# Autodesk Inventor assembly: -ZPanel
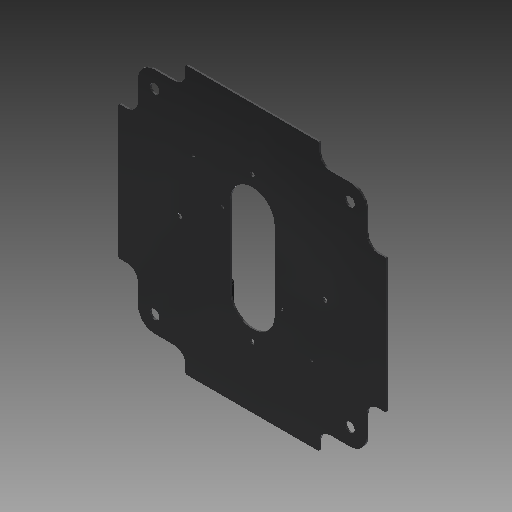
[picture p0: Inventor's stored thumbnail of the model, 512x512]
Saved by Autodesk Inventor 2018 (Build 220112000, 112)
## iProperties
Created: 2018-11-03
Part Number: -ZPanel
Document SubType Name: Assembly
Designer: Bradley
Author: Bradley
## Documents named in this file (3)
- C:\Users\Bradley\Documents\GitHub\CougSat1-Hardware\CougSat1-RadioBoard\CADModel\Native\-ZPanel.iam
- C:\Users\Bradley\Documents\GitHub\CougSat1-Hardware\CougSat1-RadioBoard\CADModel\Native\-ZPanel_PCB.ipt
- C:\Users\Bradley\Documents\GitHub\Resources\SupplierDocuments\04 - Connectors SMT\04-0001\04-0001.iam
## Components (2 placed, 2 different names)
1. 04-0001:1 [sub-assembly] — Mate:6, Mate:7, Flush:6
2. -ZPanel_PCB:1 — Mate:6
## Relationships (3: Mate 2, Flush 1)
- Mate:6: 04-0001:1 ↔ -ZPanel_PCB:1
- Mate:7 (-14 mm): 04-0001:1
- Flush:6 (20 mm): 04-0001:1
